# Autodesk Inventor assembly: DriveChain2
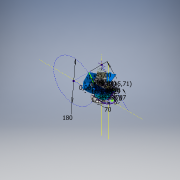
[picture p0: Inventor's stored thumbnail of the model, 180x180]
Saved by Autodesk Inventor 2018.3 (Build 223284000, 284)
## iProperties
Created: 2018-07-27
Part Number: DriveChain2
Material: Generisch
Document SubType Name: Assembly
Designer: JochenAlt
Author: JochenAlt
## Documents named in this file (12)
- D:\Projects\FlowerPot\CAD\DriveChain.iam
- D:\Projects\FlowerPot\CAD\Motor.iam
- C:\Users\JochenAlt\Documents\Inventor\Content Center Files\R2018\de-DE\DIN BEARING(1)\DIN 625 SKF - SKF 623.ipt
- D:\Projects\FlowerPot\CAD\HarmonicDrive-Axis.ipt
- D:\Projects\FlowerPot\CAD\BushOmniWheel.ipt
- D:\Projects\FlowerPot\CAD\OmniWheel-66mm.ipt
- D:\Projects\FlowerPot\CAD\Mounting Hub.ipt
- D:\Projects\FlowerPot\CAD\Encoder\Avago Encoder.iam
- D:\Projects\FlowerPot\CAD\DriveChainEnclosure2.ipt
- D:\Projects\FlowerPot\CAD\Spindle\SpindleThread.ipt
- C:\Users\JochenAlt\Documents\Inventor\Content Center Files\R2018\de-DE\DIN BEARING(1)\DIN 625 SKF - SKF 619_4.ipt
- D:\Projects\FlowerPot\CAD\Beltdrive\BeltDrive.iam
## Components (13 placed, 11 different names)
1. Motor:1 [sub-assembly] — Passend:44, Passend:53, Passend:55
2. DIN 625 SKF SKF 619/4:2 — Passend:33, Passend:46, Passend:56
3. HarmonicDrive-Axis:1 — Passend:11, Passend:13, Drehung:4, Passend:15, Passend:30, Passend:33
4. DIN 625 SKF SKF 619/4:1 — Passend:12, Passend:40, Passend:41
5. BushOmniWheel:1 — Passend:11, Passend:12, Passend:14
6. OmniWheel:1 — Passend:15, Passend:16, Drehung:6
7. Mounting Hub:1 — Passend:13, Drehung:4, Passend:14, Passend:16, Drehung:6
8. Avago Encoder:1 [sub-assembly] — Winkel:1, Passend:57
9. DriveChainEnclosure:1 — Passend:30, Passend:40, Passend:41, Passend:44, Passend:46, Passend:51, Passend:52, Passend:57
10. DIN 625 SKF SKF 623:5
11. DIN 625 SKF SKF 623:4
12. SpindleThread:1 — Passend:51, Passend:52
13. BeltDriveTest:1 [sub-assembly] — Passend:53, Passend:54, Passend:55, Passend:56
## Relationships (22: Mate 19, RelateRotation 2, Angle 1)
- Passend:11 [Mate]: HarmonicDrive-Axis:1 ↔ BushOmniWheel:1
- Passend:12 [Mate]: DIN 625 SKF SKF 619/4:1 ↔ BushOmniWheel:1
- Passend:13 [Mate]: HarmonicDrive-Axis:1 ↔ Mounting Hub:1
- Drehung:4 [RelateRotation] (-1 ul): HarmonicDrive-Axis:1 ↔ Mounting Hub:1
- Passend:14 [Mate]: BushOmniWheel:1 ↔ Mounting Hub:1
- Passend:15 [Mate]: HarmonicDrive-Axis:1 ↔ OmniWheel:1
- Passend:16 [Mate]: OmniWheel:1 ↔ Mounting Hub:1
- Drehung:6 [RelateRotation] (1 ul): OmniWheel:1 ↔ Mounting Hub:1
- Passend:30 [Mate]: HarmonicDrive-Axis:1 ↔ DriveChainEnclosure:1
- Passend:33 [Mate]: DIN 625 SKF SKF 619/4:2 ↔ HarmonicDrive-Axis:1
- Winkel:1 [Angle] (0 deg): Avago Encoder:1
- Passend:40 [Mate]: DIN 625 SKF SKF 619/4:1 ↔ DriveChainEnclosure:1
- Passend:41 [Mate]: DIN 625 SKF SKF 619/4:1 ↔ DriveChainEnclosure:1
- Passend:44 [Mate]: Motor:1 ↔ DriveChainEnclosure:1
- Passend:46 [Mate]: DIN 625 SKF SKF 619/4:2 ↔ DriveChainEnclosure:1
- Passend:51 [Mate]: DriveChainEnclosure:1 ↔ SpindleThread:1
- Passend:52 [Mate]: DriveChainEnclosure:1 ↔ SpindleThread:1
- Passend:53 [Mate]: Motor:1 ↔ BeltDriveTest:1
- Passend:54 [Mate]: BeltDriveTest:1
- Passend:55 [Mate] (0.5 mm): Motor:1 ↔ BeltDriveTest:1
- Passend:56 [Mate] (5 mm): DIN 625 SKF SKF 619/4:2 ↔ BeltDriveTest:1
- Passend:57 [Mate]: Avago Encoder:1 ↔ DriveChainEnclosure:1
